# Autodesk Inventor assembly: Ventosa
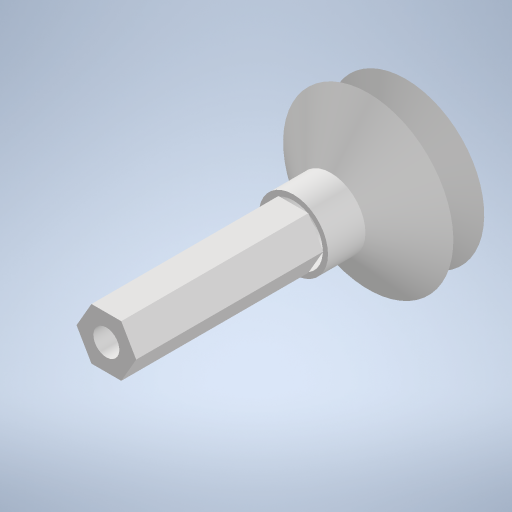
[picture p0: Inventor's stored thumbnail of the model, 512x512]
Saved by Autodesk Inventor 2023.1 (Build 271208000, 208)
## iProperties
Created: 2022-11-04
Part Number: Ventosa
Document SubType Name: Assembly
Designer: Daniel Peña
Author: Daniel Peña
## Documents named in this file (3)
- C:\Users\danie\Documents\UN\ProyectoRobotica\CAD\PortaHerramienta\Ventosa.iam
- C:\Users\danie\Documents\UN\ProyectoRobotica\CAD\PortaHerramienta\Ventosa.ipt
- C:\Users\danie\Documents\UN\ProyectoRobotica\CAD\PortaHerramienta\Montaje Manguera.ipt
## Components (2 placed, 2 different names)
1. Ventosa:1 — Mate:1, Mate:2
2. Montaje Manguera:1 — Mate:1, Mate:2
## Relationships (2: Mate 2)
- Mate:1: Ventosa:1 ↔ Montaje Manguera:1
- Mate:2: Ventosa:1 ↔ Montaje Manguera:1
